# Autodesk Inventor assembly: zlozenie
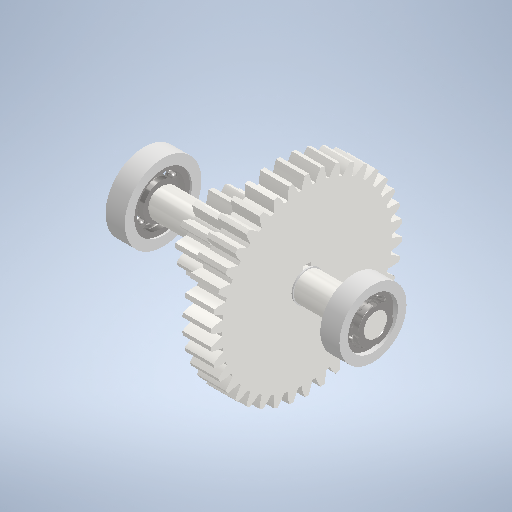
[picture p0: Inventor's stored thumbnail of the model, 512x512]
Saved by Autodesk Inventor 2025 (Build 290162000, 162)
## iProperties
Created: 2024-06-15
Part Number: zlozenie
Document SubType Name: Assembly
Designer: wikto
Author: wikto
## Documents named in this file (11)
- C:\Users\wikto\OneDrive\Pulpit\invent\zlozenie.iam
- C:\Users\wikto\OneDrive\Pulpit\invent\Wał1.ipt
- C:\Users\wikto\OneDrive\Pulpit\invent\kol\Design Accelerator\zebatka_mala.ipt
- C:\Users\wikto\OneDrive\Pulpit\invent\zlozenie\Design Accelerator\Łożysko1.iam
- C:\Users\wikto\OneDrive\Pulpit\invent\zlozenie\Design Accelerator\Łożysko2.iam
- C:\Users\wikto\OneDrive\Pulpit\invent\zebatka_duza.ipt
- C:\Users\wikto\OneDrive\Pulpit\invent\pierscien_zab_ok.ipt
- C:\Users\wikto\OneDrive\Dokumenty\Inventor\Content Center Files\R2025\pl-PL\DIN 981\DIN 981 - KM 5.ipt
- C:\Users\wikto\OneDrive\Dokumenty\Inventor\Content Center Files\R2025\pl-PL\DIN 5406 Type MB_MBL (- DIN 981)\DIN 5406 - MB5.ipt
- C:\Users\wikto\OneDrive\Pulpit\invent\korpus1.ipt
- C:\Users\wikto\OneDrive\Pulpit\invent\korpus2.ipt
## Components (13 placed, 9 different names)
1. Przekładnia walcowa1:1 — Zestawiające:1
2. Łożysko:1 [sub-assembly] — Zestawiające:4
3. Łożysko:2 [sub-assembly] — Zestawiające:5
4. Przekładnia walcowa2:1 — Zestawiające:2
5. pierscien_zab_ok:1 — Zestawiające:3
6. pierscien_zab_ok:2 — Zestawiające:6
7. DIN 981 KM 5:1 — Zestawiające:10
8. DIN 981 KM 5:3 — Zestawiające:9
9. DIN 5406 Typ MB/MBL (->DIN 981) MB5:1 — Zestawiające:8
10. DIN 5406 Typ MB/MBL (->DIN 981) MB5:2 — Zestawiające:7
11. Wał:2 — Zestawiające:1, Zestawiające:2, Zestawiające:3, Zestawiające:4, Zestawiające:5, Zestawiające:6, Zestawiające:7, Zestawiające:8, Zestawiające:9, Zestawiające:10, Zestawiające:11, Zestawiające:12
12. korpus1:1 — Zestawiające:11
13. korpus2:1 — Zestawiające:12
## Relationships (12: Mate 12)
- Zestawiające:1 [Mate]: Przekładnia walcowa1:1 ↔ Wał:2
- Zestawiające:2 [Mate]: Przekładnia walcowa2:1 ↔ Wał:2
- Zestawiające:3 [Mate]: pierscien_zab_ok:1 ↔ Wał:2
- Zestawiające:4 [Mate]: Łożysko:1 ↔ Wał:2
- Zestawiające:5 [Mate]: Łożysko:2 ↔ Wał:2
- Zestawiające:6 [Mate]: pierscien_zab_ok:2 ↔ Wał:2
- Zestawiające:7 [Mate]: DIN 5406 Typ MB/MBL (->DIN 981) MB5:2 ↔ Wał:2
- Zestawiające:8 [Mate]: DIN 5406 Typ MB/MBL (->DIN 981) MB5:1 ↔ Wał:2
- Zestawiające:9 [Mate]: DIN 981 KM 5:3 ↔ Wał:2
- Zestawiające:10 [Mate]: DIN 981 KM 5:1 ↔ Wał:2
- Zestawiające:11 [Mate]: Wał:2 ↔ korpus1:1
- Zestawiające:12 [Mate]: Wał:2 ↔ korpus2:1
